# Autodesk Inventor assembly: 2
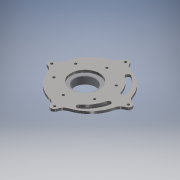
[picture p0: Inventor's stored thumbnail of the model, 180x180]
Saved by Autodesk Inventor 2019 (Build 230136000, 136)
## iProperties
Created: 2018-12-09
Part Number: 2
Document SubType Name: Assembly
Description: Large Eccentric Chain Tensioner
Material_size: As Specified
Quantity: 1
Author: steelen
## Documents named in this file (4)
- P:\me_fsae\2018_2019\ME\DriveTrain\Diff Parts\LargeEccentricChainTensioner.iam
- P:\me_fsae\2018_2019\ME\DriveTrain\Diff Parts\5972K367_BALL BEARING.ipt
- P:\me_fsae\2018_2019\ME\DriveTrain\Diff Parts\LargeBearingPlate.ipt
- P:\me_fsae\2018_2019\ME\DriveTrain\Diff Parts\LargeBearingRing.ipt
## Components (3 placed, 3 different names)
1. 5972K367_BALL BEARING:1 — Mate:1, Mate:2
2. LargeBearingPlate:1 — Insert:1, Insert:2, Mate:1
3. LargeBearingRing:1 — Insert:1, Insert:2, Mate:2
## Relationships (4: Insert 2, Mate 2)
- Insert:1: LargeBearingPlate:1 ↔ LargeBearingRing:1
- Insert:2: LargeBearingPlate:1 ↔ LargeBearingRing:1
- Mate:1: 5972K367_BALL BEARING:1 ↔ LargeBearingPlate:1
- Mate:2: 5972K367_BALL BEARING:1 ↔ LargeBearingRing:1
